# Autodesk Inventor assembly: 4.1h_JulianR_Assemblypart3
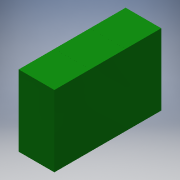
[picture p0: Inventor's stored thumbnail of the model, 180x180]
Saved by Autodesk Inventor 2016 (Build 200138000, 138)
## iProperties
Created: 2017-03-02
Part Number: 4.1h_JulianR_Assemblypart3
Document SubType Name: Assembly
Designer: fhs-mgr
Author: fhs-mgr
## Documents named in this file (2)
- H:\IED 5th Inventor\4.1h_JulianR_Assemblypart3.iam
- H:\IED 5th Inventor\WoodenBlock.ipt
## Components (6 placed, 1 different names)
1. WoodenBlock:1 — Mate:1, Mate:2
2. WoodenBlock:3 — Mate:1, Mate:2, Mate:11, Mate:12
3. WoodenBlock:4 — Mate:5, Mate:6, Mate:9, Mate:10, Flush:9, Flush:10, Flush:11, Flush:12, Flush:14, Flush:15, Flush:16
4. WoodenBlock:6 — Mate:5, Mate:6, Mate:8, Flush:8, Flush:10, Flush:11, Flush:12, Flush:13, Flush:15, Flush:17, Mate:11, Mate:12
5. WoodenBlock:7 — Mate:7, Flush:1, Flush:2, Flush:3, Flush:4, Flush:5, Flush:6, Flush:7, Mate:9, Mate:10, Flush:9, Flush:14, Flush:16, Flush:18
6. WoodenBlock:8 — Mate:7, Flush:1, Flush:2, Flush:3, Flush:4, Flush:5, Flush:6, Flush:7, Mate:8, Flush:8, Flush:13, Flush:17, Flush:18
## Relationships (28: Flush 18, Mate 10)
- Mate:1: WoodenBlock:1 ↔ WoodenBlock:3
- Mate:2: WoodenBlock:1 ↔ WoodenBlock:3
- Mate:5: WoodenBlock:4 ↔ WoodenBlock:6
- Mate:6: WoodenBlock:4 ↔ WoodenBlock:6
- Mate:7: WoodenBlock:7 ↔ WoodenBlock:8
- Flush:1: WoodenBlock:7 ↔ WoodenBlock:8
- Flush:2: WoodenBlock:7 ↔ WoodenBlock:8
- Flush:3: WoodenBlock:7 ↔ WoodenBlock:8
- Flush:4: WoodenBlock:7 ↔ WoodenBlock:8
- Flush:5: WoodenBlock:7 ↔ WoodenBlock:8
- Flush:6: WoodenBlock:7 ↔ WoodenBlock:8
- Flush:7: WoodenBlock:7 ↔ WoodenBlock:8
- Mate:8: WoodenBlock:6 ↔ WoodenBlock:8
- Mate:9: WoodenBlock:4 ↔ WoodenBlock:7
- Mate:10: WoodenBlock:4 ↔ WoodenBlock:7
- Flush:8: WoodenBlock:6 ↔ WoodenBlock:8
- Flush:9: WoodenBlock:4 ↔ WoodenBlock:7
- Flush:10: WoodenBlock:4 ↔ WoodenBlock:6
- Flush:11: WoodenBlock:4 ↔ WoodenBlock:6
- Flush:12: WoodenBlock:4 ↔ WoodenBlock:6
- Flush:13: WoodenBlock:6 ↔ WoodenBlock:8
- Flush:14: WoodenBlock:4 ↔ WoodenBlock:7
- Flush:15: WoodenBlock:4 ↔ WoodenBlock:6
- Flush:16: WoodenBlock:4 ↔ WoodenBlock:7
- Flush:17: WoodenBlock:6 ↔ WoodenBlock:8
- Flush:18: WoodenBlock:7 ↔ WoodenBlock:8
- Mate:11: WoodenBlock:3 ↔ WoodenBlock:6
- Mate:12: WoodenBlock:3 ↔ WoodenBlock:6
